# Autodesk Inventor assembly: Pistone scarico - Taglio
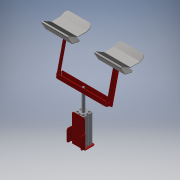
[picture p0: Inventor's stored thumbnail of the model, 180x180]
Saved by Autodesk Inventor 2018 (Build 220112000, 112)
## iProperties
Created: 2020-06-13
Part Number: Pistone scarico - Taglio
Material: Generico
Document SubType Name: Weldment
Designer: Francesco
Weld Material: Welded Aluminum-6061
Author: Francesco
## Documents named in this file (7)
- C:\Users\Francesco\no-brim\Meccanica\Progetto Inventor no-brim\Assiemi\Pistone scarico - Taglio.iam
- C:\Users\Francesco\no-brim\Meccanica\Progetto Inventor no-brim\Parti\ADN 16 - 50 A-P-A #536331\AIS2017\536331 ADN-16-50-A-P-A---(asm_0).iam
- C:\Users\Francesco\no-brim\Meccanica\Progetto Inventor no-brim\Parti\Supporto pistone scarico.ipt
- C:\Users\Francesco\no-brim\Meccanica\Progetto Inventor no-brim\Parti\Lamiera mobile pistone scarico.ipt
- C:\Users\Francesco\no-brim\Meccanica\Progetto Inventor no-brim\Parti\Lamiera pistone scarico.ipt
- C:\Users\Francesco\no-brim\Meccanica\Progetto Inventor no-brim\Parti\Lamiera scarico tubo.ipt
- C:\Users\Francesco\no-brim\Meccanica\Progetto Inventor no-brim\Parti\Lamiera pistone scarico 2.ipt
## Components (7 placed, 6 different names)
1. 536331 ADN-16-50-A-P-A---(asm_0):1 [sub-assembly] — Coincidente:1, Coincidente:2, Coincidente:3, Coincidente:4, Coincidente:5, Angolo:1, Angolo:3
2. Supporto pistone pinza:1 — Coincidente:1, Coincidente:2, Coincidente:3
3. Lamiera mobile pistone scarico:1 — Coincidente:4, Coincidente:5, Angolo:1, Coincidente:6, Coincidente:7, Coincidente:10, Coincidente:11
4. Lamiera scarico tubo:1 — Angolo:3, Coincidente:8, Coincidente:9
5. Lamiera scarico tubo:2 — Coincidente:12, Coincidente:13, Angolo:4
6. Lamiera pistone scarico:1 — Coincidente:6, Coincidente:7, Coincidente:8, Coincidente:9, Allineato:1
7. Lamiera pistone scarico 2:1 — Coincidente:10, Coincidente:11, Coincidente:12, Coincidente:13, Angolo:4, Allineato:1
## Relationships (17: Mate 13, Angle 3, Flush 1)
- Coincidente:1 [Mate]: 536331 ADN-16-50-A-P-A---(asm_0):1 ↔ Supporto pistone pinza:1
- Coincidente:2 [Mate]: 536331 ADN-16-50-A-P-A---(asm_0):1 ↔ Supporto pistone pinza:1
- Coincidente:3 [Mate]: 536331 ADN-16-50-A-P-A---(asm_0):1 ↔ Supporto pistone pinza:1
- Coincidente:4 [Mate]: 536331 ADN-16-50-A-P-A---(asm_0):1 ↔ Lamiera mobile pistone scarico:1
- Coincidente:5 [Mate]: 536331 ADN-16-50-A-P-A---(asm_0):1 ↔ Lamiera mobile pistone scarico:1
- Angolo:1 [Angle] (0 deg): 536331 ADN-16-50-A-P-A---(asm_0):1 ↔ Lamiera mobile pistone scarico:1
- Angolo:3 [Angle] (0 deg): 536331 ADN-16-50-A-P-A---(asm_0):1 ↔ Lamiera scarico tubo:1
- Coincidente:6 [Mate]: Lamiera mobile pistone scarico:1 ↔ Lamiera pistone scarico:1
- Coincidente:7 [Mate]: Lamiera mobile pistone scarico:1 ↔ Lamiera pistone scarico:1
- Coincidente:8 [Mate]: Lamiera scarico tubo:1 ↔ Lamiera pistone scarico:1
- Coincidente:9 [Mate]: Lamiera scarico tubo:1 ↔ Lamiera pistone scarico:1
- Coincidente:10 [Mate]: Lamiera mobile pistone scarico:1 ↔ Lamiera pistone scarico 2:1
- Coincidente:11 [Mate]: Lamiera mobile pistone scarico:1 ↔ Lamiera pistone scarico 2:1
- Coincidente:12 [Mate]: Lamiera scarico tubo:2 ↔ Lamiera pistone scarico 2:1
- Coincidente:13 [Mate]: Lamiera scarico tubo:2 ↔ Lamiera pistone scarico 2:1
- Angolo:4 [Angle] (0 deg): Lamiera scarico tubo:2 ↔ Lamiera pistone scarico 2:1
- Allineato:1 [Flush]: Lamiera pistone scarico:1 ↔ Lamiera pistone scarico 2:1
